# Autodesk Inventor assembly: CaseB
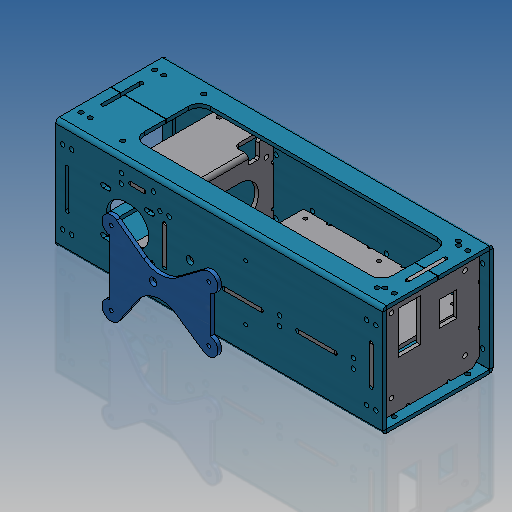
[picture p0: Inventor's stored thumbnail of the model, 512x512]
Saved by Autodesk Inventor 2017 (Build 210142000, 142)
## iProperties
Part Number: CaseB
Material: Genérico
Document SubType Name: Assembly
Designer: Leo
Author: Leo
## Documents named in this file (7)
- C:\Users\Leo\Documents\GitHub\actor-re-actor\models\inventor-caja\Case\CaseB.iam
- C:\Users\Leo\Documents\GitHub\actor-re-actor\models\inventor-caja\Case\Protector.ipt
- C:\Users\Leo\Documents\GitHub\actor-re-actor\models\inventor-caja\Case\CaseB.ipt
- C:\Users\Leo\Documents\GitHub\actor-re-actor\models\inventor-caja\Case\Refuerzo U.ipt
- C:\Users\Leo\Documents\GitHub\actor-re-actor\models\inventor-caja\Case\bandeja central.ipt
- C:\Users\Leo\Documents\GitHub\actor-re-actor\models\inventor-caja\Case\Tapa Enchufes.ipt
- C:\Users\Leo\Documents\GitHub\actor-re-actor\models\inventor-caja\Case\Pieza4.ipt
## Components (6 placed, 6 different names)
1. CaseB:1 — Coincidencia:1, Nivelación:5, Nivelación:6, Nivelación:7, Coincidencia:2, Nivelación:8, Nivelación:10, Nivelación:11, Nivelación:13
2. Protector:1 — Nivelación:1, Nivelación:2, Nivelación:3
3. Refuerzo U:1 — Nivelación:4, Coincidencia:1, Nivelación:5
4. bandeja central:1 — Nivelación:6, Nivelación:7, Coincidencia:2
5. Tapa Enchufes:1 — Nivelación:8, Nivelación:9, Nivelación:10
6. Pieza4:1 — Nivelación:11, Nivelación:12, Nivelación:13
## Relationships (15: Flush 13, Mate 2)
- Nivelación:1 [Flush] (40 mm): Protector:1
- Nivelación:2 [Flush]: Protector:1
- Nivelación:3 [Flush]: Protector:1
- Nivelación:4 [Flush]: Refuerzo U:1
- Coincidencia:1 [Mate]: CaseB:1 ↔ Refuerzo U:1
- Nivelación:5 [Flush]: CaseB:1 ↔ Refuerzo U:1
- Nivelación:6 [Flush]: CaseB:1 ↔ bandeja central:1
- Nivelación:7 [Flush]: CaseB:1 ↔ bandeja central:1
- Coincidencia:2 [Mate]: CaseB:1 ↔ bandeja central:1
- Nivelación:8 [Flush]: CaseB:1 ↔ Tapa Enchufes:1
- Nivelación:9 [Flush]: Tapa Enchufes:1
- Nivelación:10 [Flush]: CaseB:1 ↔ Tapa Enchufes:1
- Nivelación:11 [Flush]: CaseB:1 ↔ Pieza4:1
- Nivelación:12 [Flush]: Pieza4:1
- Nivelación:13 [Flush]: CaseB:1 ↔ Pieza4:1
